# Autodesk Inventor assembly: Assembly3
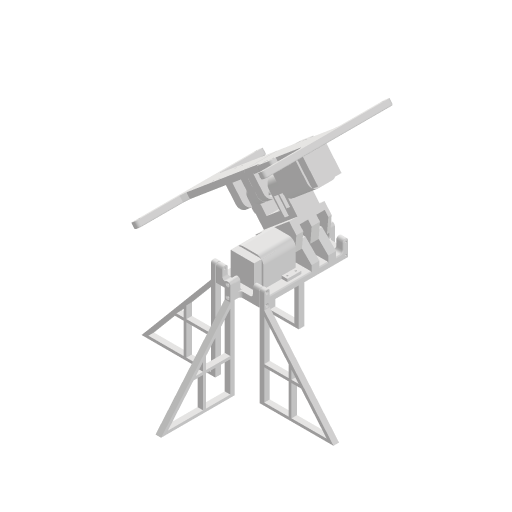
[picture p0: Inventor's stored thumbnail of the model, 512x512]
Saved by Autodesk Inventor 2023 (Build 270158000, 158)
## iProperties
Created: 2023-10-18
Part Number: Assembly3
Document SubType Name: Assembly
Designer: MVeszpremi
Author: MVeszpremi
## Documents named in this file (10)
- C:\Users\veszp\Dropbox\M202_Project\CAD\Assembly3.iam
- C:\Users\veszp\Dropbox\M202_Project\CAD\PanelBarcket.ipt
- C:\Users\veszp\Dropbox\M202_Project\CAD\StepperMotorHolder.ipt
- C:\Users\veszp\Dropbox\M202_Project\CAD\PanelBarcket_2.ipt
- C:\Users\veszp\Dropbox\M202_Project\CAD\Bearing_mount.ipt
- C:\Users\veszp\Dropbox\M202_Project\CAD\Gimbal_1.ipt
- C:\Users\veszp\Dropbox\180DAB CAD\gearedNema17.ipt
- C:\Users\veszp\Dropbox\M202_Project\CAD\Gimbal_2.ipt
- C:\Users\veszp\Dropbox\M202_Project\CAD\Base.ipt
- C:\Users\veszp\Dropbox\M202_Project\CAD\legs.ipt
## Components (14 placed, 9 different names)
1. PanelBarcket:1 — Mate:1, Mate:2, Mate:3, Mate:6, Mate:7, Mate:8, Mate:22
2. StepperMotorHolder:1 — Mate:1, Mate:2, Mate:3, Mate:11, Mate:12, Angle:1
3. PanelBarcket_2:1 — Mate:4, Mate:5, Mate:6, Mate:7, Mate:8, Mate:21, Angle:3
4. Bearing_mount:1 — Mate:4, Mate:5
5. Gimbal_1:1 — Mate:13, Mate:14, Mate:21, Mate:22, Angle:3
6. gearedNema17:1 — Mate:11, Mate:12, Angle:1
7. Gimbal_2:1 — Mate:13, Mate:14, Mate:15, Mate:20, Angle:4
8. gearedNema17:2 — Mate:15, Mate:18, Mate:19, Angle:2
9. StepperMotorHolder:2 — Mate:16, Mate:17, Mate:18, Mate:19, Angle:2, Mate:20
10. Base:1 — Mate:16, Mate:17, Mate:23, Mate:24, Mate:25, Angle:4, Mate:26, Mate:27, Mate:28, Mate:29, Mate:30, Mate:31, Mate:32
11. legs:1 — Mate:23, Mate:24, Mate:25
12. legs:2 — Mate:26, Mate:27, Mate:28
13. legs:5 — Mate:31, Mate:32
14. legs:6 — Mate:29, Mate:30
## Relationships (34: Mate 30, Angle 4)
- Mate:1: PanelBarcket:1 ↔ StepperMotorHolder:1
- Mate:2: PanelBarcket:1 ↔ StepperMotorHolder:1
- Mate:3: PanelBarcket:1 ↔ StepperMotorHolder:1
- Mate:4: PanelBarcket_2:1 ↔ Bearing_mount:1
- Mate:5: PanelBarcket_2:1 ↔ Bearing_mount:1
- Mate:6: PanelBarcket:1 ↔ PanelBarcket_2:1
- Mate:7: PanelBarcket:1 ↔ PanelBarcket_2:1
- Mate:8: PanelBarcket:1 ↔ PanelBarcket_2:1
- Mate:11: StepperMotorHolder:1 ↔ gearedNema17:1
- Mate:12: StepperMotorHolder:1 ↔ gearedNema17:1
- Angle:1 (0 deg): StepperMotorHolder:1 ↔ gearedNema17:1
- Mate:13: Gimbal_1:1 ↔ Gimbal_2:1
- Mate:14: Gimbal_1:1 ↔ Gimbal_2:1
- Mate:15: Gimbal_2:1 ↔ gearedNema17:2
- Mate:16: StepperMotorHolder:2 ↔ Base:1
- Mate:17: StepperMotorHolder:2 ↔ Base:1
- Mate:18: gearedNema17:2 ↔ StepperMotorHolder:2
- Mate:19: gearedNema17:2 ↔ StepperMotorHolder:2
- Angle:2 (0 deg): gearedNema17:2 ↔ StepperMotorHolder:2
- Mate:20 (0.25 mm): Gimbal_2:1 ↔ StepperMotorHolder:2
- Mate:21: PanelBarcket_2:1 ↔ Gimbal_1:1
- Mate:22 (0.5 mm): PanelBarcket:1 ↔ Gimbal_1:1
- Angle:3 (180 deg): PanelBarcket_2:1 ↔ Gimbal_1:1
- Mate:23: Base:1 ↔ legs:1
- Mate:24: Base:1 ↔ legs:1
- Mate:25: Base:1 ↔ legs:1
- Angle:4 (140 deg): Gimbal_2:1 ↔ Base:1
- Mate:26: Base:1 ↔ legs:2
- Mate:27: Base:1 ↔ legs:2
- Mate:28: Base:1 ↔ legs:2
- Mate:29: Base:1 ↔ legs:6
- Mate:30: Base:1 ↔ legs:6
- Mate:31: Base:1 ↔ legs:5
- Mate:32: Base:1 ↔ legs:5
